# Autodesk Inventor assembly: Left Side Arm Intake V2
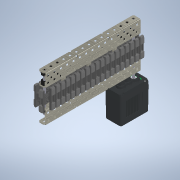
[picture p0: Inventor's stored thumbnail of the model, 180x180]
Saved by Autodesk Inventor 2020 (Build 240168000, 168)
## iProperties
Created: 2019-09-15
Part Number: Left Side Arm Intake V2
Document SubType Name: Assembly
Designer: Corey
Author: Corey
## Documents named in this file (10)
- C:\Users\Corey\Documents\Tower-Takeover-CAD\Parts\Left Side Arm Intake V2.iam
- C:\Users\Corey\Documents\Tower-Takeover-CAD\Parts\Motion\Chain & Tank Tread\Tank Tread Traction Link.ipt
- C:\Users\Corey\Documents\Tower-Takeover-CAD\Parts\Motion\Bearing Flat.ipt
- C:\Users\Corey\Documents\Tower-Takeover-CAD\Parts\Motion\Drive Shafts\Drive Shaft 4''.ipt
- C:\Users\Corey\Documents\Tower-Takeover-CAD\Parts\Electronics\V5\Smart_Motor.iam
- C:\Users\Corey\Documents\Tower-Takeover-CAD\Parts\Structure\C-Channels\Aluminum\2-Wide\Aluminum C-Channel 1x2x1x15.ipt
- C:\Users\Corey\Documents\Tower-Takeover-CAD\Parts\Motion\Drive Shafts\Drive Shaft 3''.ipt
- C:\Users\Corey\Documents\Tower-Takeover-CAD\Parts\Motion\Sprockets\High Strength 6-tooth Sprocket.ipt
- C:\Users\Corey\Documents\Tower-Takeover-CAD\Parts\Structure\Standoffs & Couplers\Standoff 1.50''.ipt
- C:\Users\Corey\Documents\Tower-Takeover-CAD\Parts\Chain Sketch for Intake.ipt
## Components (57 placed, 9 different names)
1. Bearing Flat:1 — Insert:29, Insert:30
2. Bearing Flat:2 — Insert:27, Insert:28, Insert:35
3. Bearing Flat:3 — Insert:31, Insert:32
4. Bearing Flat:5 — Insert:33, Insert:34, Insert:39
5. Drive Shaft 4'':1 — Insert:39, Mate:17, Mate:18, Flush:1
6. Smart_Motor:1 [sub-assembly] — Insert:45, Insert:46
7. Bearing Flat:6 — Insert:43, Insert:44
8. Bearing Flat:7 — Insert:23, Insert:24
9. Aluminum C-Channel 1x2x1x15:1 — Insert:23, Insert:24, Insert:40, Insert:41, Insert:42, Insert:43, Insert:44, Insert:45, Insert:46
10. Aluminum C-Channel 1x2x1x15:2 — Insert:27, Insert:28, Insert:29, Insert:30, Insert:31, Insert:32, Insert:33, Insert:34, Mate:16, Insert:36, Insert:37, Insert:38, Mate:19
11. Drive Shaft 3'':1 — Insert:35, Mate:14, Mate:15, Flush:1
12. High Strength 6-tooth Sprocket:1 — Mate:14, Mate:15, Mate:16, Mate:20, Mate:21, Mate:22, Mate:23
13. High Strength 6-tooth Sprocket:2 — Mate:17, Mate:18, Mate:19
14. Standoff 1.50'':1 — Insert:38, Insert:40
15. Standoff 1.50'':2 — Insert:37, Insert:41
16. Standoff 1.50'':3 — Insert:36, Insert:42
17. Chain Sketch for Intake:1 — Mate:20, Mate:21, Mate:22, Mate:23, Flush:2, Flush:3, Flush:4
18. Tank Tread Traction Link:1 — Flush:2, Flush:3, Flush:4
19. Tank Tread Traction Link:2
20. Tank Tread Traction Link:3
21. Tank Tread Traction Link:4
22. Tank Tread Traction Link:5
23. Tank Tread Traction Link:6
24. Tank Tread Traction Link:7
25. Tank Tread Traction Link:8
26. Tank Tread Traction Link:9
27. Tank Tread Traction Link:10
28. Tank Tread Traction Link:11
29. Tank Tread Traction Link:12
30. Tank Tread Traction Link:13
31. Tank Tread Traction Link:14
32. Tank Tread Traction Link:15
33. Tank Tread Traction Link:16
34. Tank Tread Traction Link:17
35. Tank Tread Traction Link:18
36. Tank Tread Traction Link:19
37. Tank Tread Traction Link:20
38. Tank Tread Traction Link:21
39. Tank Tread Traction Link:22
40. Tank Tread Traction Link:23
41. Tank Tread Traction Link:24
42. Tank Tread Traction Link:25
43. Tank Tread Traction Link:26
44. Tank Tread Traction Link:27
45. Tank Tread Traction Link:28
46. Tank Tread Traction Link:29
47. Tank Tread Traction Link:30
48. Tank Tread Traction Link:31
49. Tank Tread Traction Link:32
50. Tank Tread Traction Link:33
51. Tank Tread Traction Link:34
52. Tank Tread Traction Link:35
53. Tank Tread Traction Link:36
54. Tank Tread Traction Link:37
55. Tank Tread Traction Link:38
56. Tank Tread Traction Link:39
57. Tank Tread Traction Link:40
## Component patterns: (40 elements, first: Tank Tread Traction Link:1)
## Relationships (36: Insert 22, Mate 10, Flush 4)
- Insert:23: Bearing Flat:7 ↔ Aluminum C-Channel 1x2x1x15:1
- Insert:24: Bearing Flat:7 ↔ Aluminum C-Channel 1x2x1x15:1
- Insert:27: Bearing Flat:2 ↔ Aluminum C-Channel 1x2x1x15:2
- Insert:28: Bearing Flat:2 ↔ Aluminum C-Channel 1x2x1x15:2
- Insert:29: Bearing Flat:1 ↔ Aluminum C-Channel 1x2x1x15:2
- Insert:30: Bearing Flat:1 ↔ Aluminum C-Channel 1x2x1x15:2
- Insert:31: Bearing Flat:3 ↔ Aluminum C-Channel 1x2x1x15:2
- Insert:32: Bearing Flat:3 ↔ Aluminum C-Channel 1x2x1x15:2
- Insert:33: Bearing Flat:5 ↔ Aluminum C-Channel 1x2x1x15:2
- Insert:34: Bearing Flat:5 ↔ Aluminum C-Channel 1x2x1x15:2
- Insert:35: Bearing Flat:2 ↔ Drive Shaft 3'':1
- Mate:14: Drive Shaft 3'':1 ↔ High Strength 6-tooth Sprocket:1
- Mate:15: Drive Shaft 3'':1 ↔ High Strength 6-tooth Sprocket:1
- Mate:16 (12.7 mm): Aluminum C-Channel 1x2x1x15:2 ↔ High Strength 6-tooth Sprocket:1
- Insert:36: Aluminum C-Channel 1x2x1x15:2 ↔ Standoff 1.50'':3
- Insert:37: Aluminum C-Channel 1x2x1x15:2 ↔ Standoff 1.50'':2
- Insert:38: Aluminum C-Channel 1x2x1x15:2 ↔ Standoff 1.50'':1
- Insert:39: Bearing Flat:5 ↔ Drive Shaft 4'':1
- Mate:17: Drive Shaft 4'':1 ↔ High Strength 6-tooth Sprocket:2
- Mate:18: Drive Shaft 4'':1 ↔ High Strength 6-tooth Sprocket:2
- Mate:19 (12.7 mm): Aluminum C-Channel 1x2x1x15:2 ↔ High Strength 6-tooth Sprocket:2
- Insert:40: Aluminum C-Channel 1x2x1x15:1 ↔ Standoff 1.50'':1
- Insert:41: Aluminum C-Channel 1x2x1x15:1 ↔ Standoff 1.50'':2
- Insert:42: Aluminum C-Channel 1x2x1x15:1 ↔ Standoff 1.50'':3
- Insert:43: Bearing Flat:6 ↔ Aluminum C-Channel 1x2x1x15:1
- Insert:44: Bearing Flat:6 ↔ Aluminum C-Channel 1x2x1x15:1
- Insert:45: Smart_Motor:1 ↔ Aluminum C-Channel 1x2x1x15:1
- Insert:46: Smart_Motor:1 ↔ Aluminum C-Channel 1x2x1x15:1
- Flush:1: Drive Shaft 4'':1 ↔ Drive Shaft 3'':1
- Mate:20: High Strength 6-tooth Sprocket:1 ↔ Chain Sketch for Intake:1
- Mate:21: High Strength 6-tooth Sprocket:1 ↔ Chain Sketch for Intake:1
- Mate:22: High Strength 6-tooth Sprocket:1 ↔ Chain Sketch for Intake:1
- Mate:23: High Strength 6-tooth Sprocket:1 ↔ Chain Sketch for Intake:1
- Flush:2: Chain Sketch for Intake:1 ↔ Tank Tread Traction Link:1
- Flush:3 (-177.8 mm): Chain Sketch for Intake:1 ↔ Tank Tread Traction Link:1
- Flush:4 (10.16 mm): Chain Sketch for Intake:1 ↔ Tank Tread Traction Link:1
